# Autodesk Inventor assembly: Winder Assembly 1
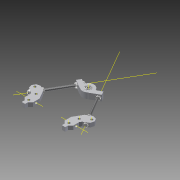
[picture p0: Inventor's stored thumbnail of the model, 180x180]
Saved by Autodesk Inventor 2013 (Build 170138000, 138)
## iProperties
Created: 2012-12-31
Part Number: Winder Assembly 1
Document SubType Name: Assembly
Designer: Nico
Mass: 167.628 g
Surface Area: 484.558 cm^2
Volume: 112.229 cm^3
Density: 1.49363 g/cm^3
Author: Nico
## Documents named in this file (8)
- D:\Documents\Inventor\Coil winder\IAM files\Winder Assembly 1.iam
- D:\Documents\Inventor\Coil winder\Drive thread.ipt
- D:\Documents\Inventor\Coil winder\IPT files\Washer M8.ipt
- D:\Documents\Inventor\Coil winder\IPT files\right top.ipt
- D:\Documents\Inventor\Coil winder\IPT files\Vertex Bottom with foot.ipt
- D:\Documents\Inventor\Coil winder\IPT files\Half Nut M8.ipt
- D:\Documents\Inventor\Coil winder\IPT files\608ZZ bearing.ipt
- D:\Documents\Inventor\Coil winder\Drive thread\Thread rod M8 x 150 mm.ipt
## Components (23 placed, 6 different names)
1. Vertex Bottom with foot:1 — Flush:1, Mate:1, Mate:3, Mate:4, Mate:36, Mate:37
2. Vertex Bottom with foot:2 — Flush:1, Mate:1, Mate:2, Mate:5, Mate:24, Mate:25
3. right top:1 — Mate:2, Mate:3, Mate:20, Mate:21, Mate:30, Mate:32, Mate:33, Mate:38, Mate:39, Mate:40, Mate:41
4. Thread rod M8 x 150 mm:1 — Mate:5, Mate:18, Mate:19, Mate:22, Mate:23, Flush:2, Flush:3
5. Thread rod M8 x 150 mm:2 — Mate:4, Mate:31, Mate:34, Mate:35, Flush:4, Flush:5
6. Washer M8:1 — Mate:7, Mate:16, Mate:20
7. Washer M8:2 — Mate:6, Mate:17, Mate:18, Mate:21
8. Washer M8:3 — Mate:8, Mate:14, Mate:24
9. Washer M8:4 — Mate:9, Mate:15, Mate:25
10. Washer M8:5 — Mate:10, Mate:29, Mate:37
11. Washer M8:6 — Mate:11, Mate:28, Mate:36
12. Washer M8:7 — Mate:12, Mate:27, Mate:32
13. Washer M8:8 — Mate:13, Mate:26, Mate:33
14. Half Nut M8:1 — Mate:10, Mate:29, Mate:35
15. Half Nut M8:2 — Mate:11, Mate:28, Mate:34, Flush:4
16. Half Nut M8:3 — Mate:12, Mate:27, Mate:31, Flush:5
17. Half Nut M8:4 — Mate:13, Mate:26, Mate:30
18. Half Nut M8:5 — Mate:6, Mate:17, Flush:3
19. Half Nut M8:6 — Mate:7, Mate:16, Mate:19
20. Half Nut M8:7 — Mate:8, Mate:14, Mate:22
21. Half Nut M8:8 — Mate:9, Mate:15, Mate:23, Flush:2
22. 608ZZ bearing:1 — Mate:38, Mate:41
23. 608ZZ bearing:2 — Mate:39, Mate:40
## Relationships (46: Mate 41, Flush 5)
- Flush:1: Vertex Bottom with foot:1 ↔ Vertex Bottom with foot:2
- Mate:1: Vertex Bottom with foot:1 ↔ Vertex Bottom with foot:2
- Mate:2: Vertex Bottom with foot:2 ↔ right top:1
- Mate:3: Vertex Bottom with foot:1 ↔ right top:1
- Mate:4: Vertex Bottom with foot:1 ↔ Thread rod M8 x 150 mm:2
- Mate:5: Vertex Bottom with foot:2 ↔ Thread rod M8 x 150 mm:1
- Mate:6: Washer M8:2 ↔ Half Nut M8:5
- Mate:7: Washer M8:1 ↔ Half Nut M8:6
- Mate:8: Washer M8:3 ↔ Half Nut M8:7
- Mate:9: Washer M8:4 ↔ Half Nut M8:8
- Mate:10: Washer M8:5 ↔ Half Nut M8:1
- Mate:11: Washer M8:6 ↔ Half Nut M8:2
- Mate:12: Washer M8:7 ↔ Half Nut M8:3
- Mate:13: Washer M8:8 ↔ Half Nut M8:4
- Mate:14: Washer M8:3 ↔ Half Nut M8:7
- Mate:15: Washer M8:4 ↔ Half Nut M8:8
- Mate:16: Washer M8:1 ↔ Half Nut M8:6
- Mate:17: Washer M8:2 ↔ Half Nut M8:5
- Mate:18: Thread rod M8 x 150 mm:1 ↔ Washer M8:2
- Mate:19: Thread rod M8 x 150 mm:1 ↔ Half Nut M8:6
- Mate:20: right top:1 ↔ Washer M8:1
- Mate:21: right top:1 ↔ Washer M8:2
- Mate:22: Thread rod M8 x 150 mm:1 ↔ Half Nut M8:7
- Mate:23: Thread rod M8 x 150 mm:1 ↔ Half Nut M8:8
- Mate:24: Vertex Bottom with foot:2 ↔ Washer M8:3
- Mate:25: Vertex Bottom with foot:2 ↔ Washer M8:4
- Flush:2 (-2 mm): Thread rod M8 x 150 mm:1 ↔ Half Nut M8:8
- Flush:3 (-2 mm): Thread rod M8 x 150 mm:1 ↔ Half Nut M8:5
- Mate:26: Washer M8:8 ↔ Half Nut M8:4
- Mate:27: Washer M8:7 ↔ Half Nut M8:3
- Mate:28: Washer M8:6 ↔ Half Nut M8:2
- Mate:29: Washer M8:5 ↔ Half Nut M8:1
- Mate:30: right top:1 ↔ Half Nut M8:4
- Mate:31: Thread rod M8 x 150 mm:2 ↔ Half Nut M8:3
- Mate:32: right top:1 ↔ Washer M8:7
- Mate:33: right top:1 ↔ Washer M8:8
- Mate:34: Thread rod M8 x 150 mm:2 ↔ Half Nut M8:2
- Mate:35: Thread rod M8 x 150 mm:2 ↔ Half Nut M8:1
- Mate:36: Vertex Bottom with foot:1 ↔ Washer M8:6
- Mate:37: Vertex Bottom with foot:1 ↔ Washer M8:5
- Flush:4 (2 mm): Thread rod M8 x 150 mm:2 ↔ Half Nut M8:2
- Flush:5 (-2 mm): Thread rod M8 x 150 mm:2 ↔ Half Nut M8:3
- Mate:38: right top:1 ↔ 608ZZ bearing:1
- Mate:39: right top:1 ↔ 608ZZ bearing:2
- Mate:40: right top:1 ↔ 608ZZ bearing:2
- Mate:41: right top:1 ↔ 608ZZ bearing:1
